# Autodesk Inventor assembly: Conjunto
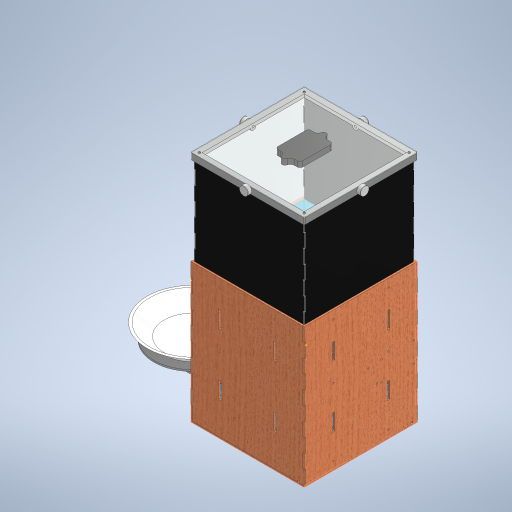
[picture p0: Inventor's stored thumbnail of the model, 512x512]
Saved by Autodesk Inventor 2024.2 (Build 282272000, 272)
## iProperties
Created: 2024-07-16
Part Number: Conjunto
Document SubType Name: Assembly
Designer: sergi
Author: sergi
## Documents named in this file (35)
- C:\Users\sergi\OneDrive\Escritorio\Projects\Automatic Feeder\ComederoV6\Inventor\Conjunto.iam
- C:\Users\sergi\OneDrive\Escritorio\Projects\Automatic Feeder\ComederoV6\Inventor\Contenedor.ipt
- C:\Users\sergi\OneDrive\Escritorio\Projects\Automatic Feeder\ComederoV6\Inventor\Contenedor_Pared_1.ipt
- C:\Users\sergi\OneDrive\Escritorio\Projects\Automatic Feeder\ComederoV6\Inventor\Tolva.ipt
- C:\Users\sergi\OneDrive\Escritorio\Projects\Automatic Feeder\ComederoV6\Inventor\Rodamiento.ipt
- C:\Users\sergi\OneDrive\Escritorio\Projects\Automatic Feeder\ComederoV6\Inventor\Brida_Rodamiento.ipt
- C:\Users\sergi\OneDrive\Escritorio\Projects\Automatic Feeder\ComederoV6\Inventor\Celda_Carga.ipt
- C:\Users\sergi\OneDrive\Escritorio\Projects\Automatic Feeder\ComederoV6\Inventor\Envolvente.ipt
- C:\Users\sergi\OneDrive\Escritorio\Projects\Automatic Feeder\ComederoV6\Inventor\Envolvente_Pared_1.ipt
- C:\Users\sergi\OneDrive\Escritorio\Projects\Automatic Feeder\ComederoV6\Inventor\Soporte_Dosificador.ipt
- C:\Users\sergi\OneDrive\Escritorio\Projects\Automatic Feeder\ComederoV6\Inventor\Brida_Rodamiento_Inferior.ipt
- C:\Users\sergi\OneDrive\Escritorio\Projects\Automatic Feeder\ComederoV6\Inventor\Tope_Dosificador.ipt
- C:\Users\sergi\OneDrive\Escritorio\Projects\Automatic Feeder\ComederoV6\Inventor\Contrapeso.ipt
- C:\Users\sergi\OneDrive\Escritorio\Projects\Automatic Feeder\ComederoV6\Inventor\Cemento.ipt
- C:\Users\sergi\OneDrive\Escritorio\Projects\Automatic Feeder\ComederoV6\Inventor\Tapa_Inferior.ipt
- C:\Users\sergi\OneDrive\Escritorio\Projects\Automatic Feeder\ComederoV6\Inventor\Union_Inferior.ipt
- C:\Users\sergi\OneDrive\Escritorio\Projects\Automatic Feeder\ComederoV6\Inventor\Envolvente_Pared_2.ipt
- C:\Users\sergi\OneDrive\Escritorio\Projects\Automatic Feeder\ComederoV6\Inventor\Rampa_Salida.ipt
- C:\Users\sergi\OneDrive\Escritorio\Projects\Automatic Feeder\ComederoV6\Inventor\Soporte_Cuenco.ipt
- C:\Users\sergi\OneDrive\Escritorio\Projects\Automatic Feeder\ComederoV6\Inventor\Cuenco.ipt
- C:\Users\sergi\OneDrive\Escritorio\Projects\Automatic Feeder\ComederoV6\Inventor\Base_Plato.ipt
- C:\Users\sergi\OneDrive\Escritorio\Projects\Automatic Feeder\ComederoV6\Inventor\Aspas.ipt
- C:\Users\sergi\OneDrive\Escritorio\Projects\Automatic Feeder\ComederoV6\Inventor\Tapadera.ipt
- C:\Users\sergi\OneDrive\Escritorio\Projects\Automatic Feeder\ComederoV6\Inventor\Marco_Tapa.ipt
- C:\Users\sergi\OneDrive\Escritorio\Projects\Automatic Feeder\ComederoV6\Inventor\Deshumidicador.ipt
- C:\Users\sergi\OneDrive\Escritorio\Projects\Automatic Feeder\ComederoV6\Inventor\Servomotor.ipt
- C:\Users\sergi\OneDrive\Escritorio\Projects\Automatic Feeder\ComederoV6\Inventor\Engranajes.iam
- C:\Users\sergi\OneDrive\Escritorio\Projects\Automatic Feeder\ComederoV6\Inventor\Gears\Design Accelerator\Soporte_Servo.ipt
- C:\Users\sergi\OneDrive\Escritorio\Projects\Automatic Feeder\ComederoV6\Inventor\Cabeza_Tornillos.ipt
- C:\Users\sergi\OneDrive\Escritorio\Projects\Automatic Feeder\ComederoV6\Inventor\Tapa_Cabeza_Tornillo.ipt
- C:\Users\sergi\OneDrive\Escritorio\Projects\Automatic Feeder\ComederoV6\Inventor\ESP32S3.ipt
- C:\Users\sergi\OneDrive\Escritorio\Projects\Automatic Feeder\ComederoV6\Inventor\Soporte_ESP32S3.ipt
- C:\Users\sergi\OneDrive\Escritorio\Projects\Automatic Feeder\ComederoV6\Inventor\Buck.ipt
- C:\Users\sergi\OneDrive\Escritorio\Projects\Automatic Feeder\ComederoV6\Inventor\Envolvente_Pared_Trasera.ipt
- C:\Users\sergi\OneDrive\Escritorio\Projects\Automatic Feeder\ComederoV6\Inventor\Envolvente_Pared_Derecha.ipt
## Components (59 placed, 34 different names)
1. Contenedor:1 — Nivelación:1
2. Contenedor_Pared_1:1 — Nivelación:1, Coincidencia:1, Nivelación:2, Nivelación:3, Nivelación:43
3. Contenedor_Pared_1:2 — Coincidencia:1, Nivelación:2, Nivelación:3, Nivelación:6, Coincidencia:3, Nivelación:7, Nivelación:8, Nivelación:13
4. Contenedor_Pared_1:3 — Nivelación:4, Nivelación:6, Coincidencia:3, Nivelación:7
5. Contenedor_Pared_1:4 — Nivelación:4
6. Tolva:1 — Nivelación:8, Coincidencia:4, Coincidencia:5, Nivelación:9, Coincidencia:78
7. Rodamiento:1 — Coincidencia:4, Coincidencia:5
8. Brida_Rodamiento:1 — Nivelación:9, Coincidencia:77
9. Celda_Carga:1 — Coincidencia:67, Coincidencia:70, Coincidencia:72, Coincidencia:74
10. Rodamiento:2 — Coincidencia:37
11. Envolvente:1 — Nivelación:13
12. Envolvente_Pared_1:2 — Coincidencia:13
13. Soporte_Dosificador:1 — Coincidencia:30, Coincidencia:35, Coincidencia:38, Coincidencia:39, Coincidencia:42, Coincidencia:43, Coincidencia:44, Coincidencia:45, Coincidencia:50, Coincidencia:51, Nivelación:30, Nivelación:31, Ángulo:1, Coincidencia:80, Coincidencia:81, Coincidencia:82, Coincidencia:83
14. Tope_Dosificador:1
15. Contrapeso:1 — Coincidencia:27, Coincidencia:28, Coincidencia:29, Coincidencia:33
16. Cemento:1 — Coincidencia:27, Coincidencia:28, Coincidencia:29
17. Tapa_Inferior:1 — Nivelación:27, Coincidencia:12, Coincidencia:14, Coincidencia:17, Coincidencia:18, Coincidencia:21, Coincidencia:22, Coincidencia:23, Coincidencia:24, Coincidencia:25, Coincidencia:26, Nivelación:28, Nivelación:29, Coincidencia:32, Coincidencia:33, Coincidencia:52, Coincidencia:53, Coincidencia:54, Coincidencia:55, Coincidencia:56, Coincidencia:57, Coincidencia:58, Coincidencia:59, Coincidencia:73, Ángulo:2, Coincidencia:100, Nivelación:100, Nivelación:101, Nivelación:102, Nivelación:103
18. Union_Inferior:1 — Nivelación:27
19. Union_Inferior:2 — Coincidencia:12, Coincidencia:13, Coincidencia:14
20. Union_Inferior:3 — Coincidencia:17, Coincidencia:32
21. Union_Inferior:4 — Coincidencia:18
22. Union_Inferior:5 — Coincidencia:22, Coincidencia:103
23. Union_Inferior:6 — Coincidencia:23, Coincidencia:26, Nivelación:28
24. Union_Inferior:7 — Coincidencia:21
25. Union_Inferior:8 — Coincidencia:24, Coincidencia:25, Nivelación:29
26. Brida_Rodamiento_Inferior:1 — Coincidencia:30, Coincidencia:35, Coincidencia:37
27. Union_Inferior:9 — Coincidencia:45, Coincidencia:55
28. Union_Inferior:10 — Coincidencia:51, Coincidencia:56
29. Union_Inferior:11 — Coincidencia:39, Coincidencia:53
30. Union_Inferior:12 — Coincidencia:38, Coincidencia:52, Coincidencia:97
31. Union_Inferior:13 — Coincidencia:44, Coincidencia:54
32. Union_Inferior:14 — Coincidencia:50, Coincidencia:57
33. Union_Inferior:15 — Coincidencia:42, Nivelación:31, Coincidencia:59
34. Union_Inferior:16 — Coincidencia:43, Nivelación:30, Coincidencia:58
35. Envolvente_Pared_2:1 — Nivelación:38, Nivelación:39, Nivelación:40, Coincidencia:65, Coincidencia:66, Coincidencia:73
36. Rampa_Salida:1 — Nivelación:38, Nivelación:39
37. Soporte_Cuenco:1 — Nivelación:40, Coincidencia:61, Coincidencia:72, Coincidencia:74
38. Cuenco:1 — Coincidencia:61, Coincidencia:65, Coincidencia:66, Coincidencia:67, Coincidencia:68, Coincidencia:69
39. Base_Plato:1 — Coincidencia:68, Coincidencia:69, Coincidencia:70
40. Aspas:1
41. Tapadera:1 — Coincidencia:75, Nivelación:44
42. Marco_Tapa:1 — Nivelación:43, Coincidencia:75, Coincidencia:84, Coincidencia:85, Coincidencia:86, Coincidencia:87, Coincidencia:89, Coincidencia:90, Coincidencia:91, Coincidencia:92
43. Deshumidicador:1 — Nivelación:44
44. Servomotor:1 — Coincidencia:79, Ángulo:1
45. Engranajes:1 [sub-assembly] — Coincidencia:77, Coincidencia:78, Coincidencia:79, Coincidencia:80
46. Soporte_Servo:1 — Coincidencia:81, Coincidencia:82, Coincidencia:83
47. Cabeza_Tornillos:1 — Nivelación:45, Coincidencia:84, Coincidencia:85
48. Tapa_Cabeza_Tornillo:1 — Nivelación:45
49. Cabeza_Tornillos:2 — Coincidencia:86, Coincidencia:87, Coincidencia:88
50. Tapa_Cabeza_Tornillo:2 — Coincidencia:88
51. Cabeza_Tornillos:3 — Coincidencia:91, Coincidencia:92, Coincidencia:93
52. Tapa_Cabeza_Tornillo:3 — Coincidencia:93
53. Cabeza_Tornillos:4 — Coincidencia:89, Coincidencia:90, Coincidencia:94, Coincidencia:95
54. Tapa_Cabeza_Tornillo:4 — Coincidencia:94, Coincidencia:95
55. ESP32S3:1 — Nivelación:49
56. Soporte_ESP32S3:1 — Nivelación:49, Coincidencia:97, Coincidencia:99, Nivelación:99, Coincidencia:101
57. Buck:1 — Ángulo:2, Coincidencia:99, Nivelación:99, Coincidencia:102
58. Envolvente_Pared_Trasera:1 — Coincidencia:100, Nivelación:100, Nivelación:101, Coincidencia:101, Coincidencia:102
59. Envolvente_Pared_Derecha:1 — Coincidencia:103, Nivelación:102, Nivelación:103
## Relationships (108: Mate 76, Flush 30, Angle 2)
- Nivelación:1 [Flush]: Contenedor:1 ↔ Contenedor_Pared_1:1
- Coincidencia:1 [Mate]: Contenedor_Pared_1:1 ↔ Contenedor_Pared_1:2
- Nivelación:2 [Flush]: Contenedor_Pared_1:1 ↔ Contenedor_Pared_1:2
- Nivelación:3 [Flush]: Contenedor_Pared_1:1 ↔ Contenedor_Pared_1:2
- [Mate]: Contenedor_Pared_1:3 ↔ Contenedor_Pared_1:4
- Nivelación:4 [Flush]: Contenedor_Pared_1:3 ↔ Contenedor_Pared_1:4
- [Flush]: Contenedor_Pared_1:3 ↔ Contenedor_Pared_1:4
- Nivelación:6 [Flush]: Contenedor_Pared_1:2 ↔ Contenedor_Pared_1:3
- Coincidencia:3 [Mate]: Contenedor_Pared_1:2 ↔ Contenedor_Pared_1:3
- Nivelación:7 [Flush]: Contenedor_Pared_1:2 ↔ Contenedor_Pared_1:3
- Nivelación:8 [Flush]: Contenedor_Pared_1:2 ↔ Tolva:1
- Coincidencia:4 [Mate]: Tolva:1 ↔ Rodamiento:1
- Coincidencia:5 [Mate]: Tolva:1 ↔ Rodamiento:1
- Nivelación:9 [Flush]: Tolva:1 ↔ Brida_Rodamiento:1
- Nivelación:13 [Flush]: Contenedor_Pared_1:2 ↔ Envolvente:1
- Nivelación:27 [Flush]: Tapa_Inferior:1 ↔ Union_Inferior:1
- Coincidencia:12 [Mate]: Tapa_Inferior:1 ↔ Union_Inferior:2
- Coincidencia:13 [Mate]: Envolvente_Pared_1:2 ↔ Union_Inferior:2
- Coincidencia:14 [Mate]: Tapa_Inferior:1 ↔ Union_Inferior:2
- Coincidencia:17 [Mate]: Tapa_Inferior:1 ↔ Union_Inferior:3
- Coincidencia:18 [Mate]: Tapa_Inferior:1 ↔ Union_Inferior:4
- Coincidencia:21 [Mate]: Tapa_Inferior:1 ↔ Union_Inferior:7
- Coincidencia:22 [Mate]: Tapa_Inferior:1 ↔ Union_Inferior:5
- Coincidencia:23 [Mate]: Tapa_Inferior:1 ↔ Union_Inferior:6
- Coincidencia:24 [Mate]: Tapa_Inferior:1 ↔ Union_Inferior:8
- Coincidencia:25 [Mate]: Tapa_Inferior:1 ↔ Union_Inferior:8
- Coincidencia:26 [Mate]: Tapa_Inferior:1 ↔ Union_Inferior:6
- Nivelación:28 [Flush] (3 mm): Tapa_Inferior:1 ↔ Union_Inferior:6
- Nivelación:29 [Flush] (3 mm): Tapa_Inferior:1 ↔ Union_Inferior:8
- Coincidencia:27 [Mate]: Contrapeso:1 ↔ Cemento:1
- Coincidencia:28 [Mate]: Contrapeso:1 ↔ Cemento:1
- Coincidencia:29 [Mate]: Contrapeso:1 ↔ Cemento:1
- Coincidencia:30 [Mate]: Soporte_Dosificador:1 ↔ Brida_Rodamiento_Inferior:1
- Coincidencia:32 [Mate]: Tapa_Inferior:1 ↔ Union_Inferior:3
- Coincidencia:33 [Mate]: Contrapeso:1 ↔ Tapa_Inferior:1
- Coincidencia:35 [Mate]: Soporte_Dosificador:1 ↔ Brida_Rodamiento_Inferior:1
- Coincidencia:37 [Mate]: Rodamiento:2 ↔ Brida_Rodamiento_Inferior:1
- Coincidencia:38 [Mate]: Soporte_Dosificador:1 ↔ Union_Inferior:12
- Coincidencia:39 [Mate]: Soporte_Dosificador:1 ↔ Union_Inferior:11
- Coincidencia:42 [Mate]: Soporte_Dosificador:1 ↔ Union_Inferior:15
- Coincidencia:43 [Mate]: Soporte_Dosificador:1 ↔ Union_Inferior:16
- Coincidencia:44 [Mate]: Soporte_Dosificador:1 ↔ Union_Inferior:13
- Coincidencia:45 [Mate]: Soporte_Dosificador:1 ↔ Union_Inferior:9
- Coincidencia:50 [Mate]: Soporte_Dosificador:1 ↔ Union_Inferior:14
- Coincidencia:51 [Mate]: Soporte_Dosificador:1 ↔ Union_Inferior:10
- Coincidencia:52 [Mate]: Tapa_Inferior:1 ↔ Union_Inferior:12
- Coincidencia:53 [Mate]: Tapa_Inferior:1 ↔ Union_Inferior:11
- Coincidencia:54 [Mate]: Tapa_Inferior:1 ↔ Union_Inferior:13
- Coincidencia:55 [Mate]: Tapa_Inferior:1 ↔ Union_Inferior:9
- Coincidencia:56 [Mate]: Tapa_Inferior:1 ↔ Union_Inferior:10
- Coincidencia:57 [Mate]: Tapa_Inferior:1 ↔ Union_Inferior:14
- Nivelación:30 [Flush]: Soporte_Dosificador:1 ↔ Union_Inferior:16
- Nivelación:31 [Flush]: Soporte_Dosificador:1 ↔ Union_Inferior:15
- Coincidencia:58 [Mate]: Tapa_Inferior:1 ↔ Union_Inferior:16
- Coincidencia:59 [Mate]: Tapa_Inferior:1 ↔ Union_Inferior:15
- Nivelación:38 [Flush]: Envolvente_Pared_2:1 ↔ Rampa_Salida:1
- Nivelación:39 [Flush]: Envolvente_Pared_2:1 ↔ Rampa_Salida:1
- Nivelación:40 [Flush]: Envolvente_Pared_2:1 ↔ Soporte_Cuenco:1
- Coincidencia:61 [Mate]: Soporte_Cuenco:1 ↔ Cuenco:1
- Coincidencia:65 [Mate] (100 mm): Envolvente_Pared_2:1 ↔ Cuenco:1
- Coincidencia:66 [Mate] (-103 mm): Envolvente_Pared_2:1 ↔ Cuenco:1
- Coincidencia:67 [Mate]: Celda_Carga:1 ↔ Cuenco:1
- Coincidencia:68 [Mate]: Cuenco:1 ↔ Base_Plato:1
- Coincidencia:69 [Mate]: Cuenco:1 ↔ Base_Plato:1
- Coincidencia:70 [Mate]: Celda_Carga:1 ↔ Base_Plato:1
- Coincidencia:72 [Mate] (20.05 mm): Celda_Carga:1 ↔ Soporte_Cuenco:1
- Coincidencia:73 [Mate]: Tapa_Inferior:1 ↔ Envolvente_Pared_2:1
- Coincidencia:74 [Mate]: Celda_Carga:1 ↔ Soporte_Cuenco:1
- Nivelación:43 [Flush]: Contenedor_Pared_1:1 ↔ Marco_Tapa:1
- Coincidencia:75 [Mate]: Tapadera:1 ↔ Marco_Tapa:1
- Nivelación:44 [Flush]: Tapadera:1 ↔ Deshumidicador:1
- Coincidencia:77 [Mate]: Brida_Rodamiento:1 ↔ Engranajes:1
- Coincidencia:78 [Mate] (2 mm): Tolva:1 ↔ Engranajes:1
- Coincidencia:79 [Mate]: Servomotor:1 ↔ Engranajes:1
- Ángulo:1 [Angle] (0 deg): Soporte_Dosificador:1 ↔ Servomotor:1
- Coincidencia:80 [Mate]: Soporte_Dosificador:1 ↔ Engranajes:1
- Coincidencia:81 [Mate]: Soporte_Dosificador:1 ↔ Soporte_Servo:1
- Coincidencia:82 [Mate]: Soporte_Dosificador:1 ↔ Soporte_Servo:1
- Coincidencia:83 [Mate]: Soporte_Dosificador:1 ↔ Soporte_Servo:1
- Nivelación:45 [Flush]: Cabeza_Tornillos:1 ↔ Tapa_Cabeza_Tornillo:1
- [Flush]: Cabeza_Tornillos:2 ↔ Tapa_Cabeza_Tornillo:2
- [Flush]: Cabeza_Tornillos:3 ↔ Tapa_Cabeza_Tornillo:3
- [Flush]: Cabeza_Tornillos:4 ↔ Tapa_Cabeza_Tornillo:4
- Coincidencia:84 [Mate]: Marco_Tapa:1 ↔ Cabeza_Tornillos:1
- Coincidencia:85 [Mate]: Marco_Tapa:1 ↔ Cabeza_Tornillos:1
- Coincidencia:86 [Mate]: Marco_Tapa:1 ↔ Cabeza_Tornillos:2
- Coincidencia:87 [Mate]: Marco_Tapa:1 ↔ Cabeza_Tornillos:2
- Coincidencia:88 [Mate]: Cabeza_Tornillos:2 ↔ Tapa_Cabeza_Tornillo:2
- Coincidencia:89 [Mate]: Marco_Tapa:1 ↔ Cabeza_Tornillos:4
- Coincidencia:90 [Mate]: Marco_Tapa:1 ↔ Cabeza_Tornillos:4
- Coincidencia:91 [Mate]: Marco_Tapa:1 ↔ Cabeza_Tornillos:3
- Coincidencia:92 [Mate]: Marco_Tapa:1 ↔ Cabeza_Tornillos:3
- Coincidencia:93 [Mate]: Cabeza_Tornillos:3 ↔ Tapa_Cabeza_Tornillo:3
- Coincidencia:94 [Mate]: Cabeza_Tornillos:4 ↔ Tapa_Cabeza_Tornillo:4
- Coincidencia:95 [Mate]: Cabeza_Tornillos:4 ↔ Tapa_Cabeza_Tornillo:4
- Nivelación:49 [Flush]: ESP32S3:1 ↔ Soporte_ESP32S3:1
- Coincidencia:97 [Mate] (3 mm): Union_Inferior:12 ↔ Soporte_ESP32S3:1
- Ángulo:2 [Angle] (0 deg): Tapa_Inferior:1 ↔ Buck:1
- Coincidencia:99 [Mate] (2 mm): Soporte_ESP32S3:1 ↔ Buck:1
- Nivelación:99 [Flush] (-5 mm): Soporte_ESP32S3:1 ↔ Buck:1
- Coincidencia:100 [Mate]: Tapa_Inferior:1 ↔ Envolvente_Pared_Trasera:1
- Nivelación:100 [Flush]: Tapa_Inferior:1 ↔ Envolvente_Pared_Trasera:1
- Nivelación:101 [Flush]: Tapa_Inferior:1 ↔ Envolvente_Pared_Trasera:1
- Coincidencia:101 [Mate]: Soporte_ESP32S3:1 ↔ Envolvente_Pared_Trasera:1
- Coincidencia:102 [Mate]: Buck:1 ↔ Envolvente_Pared_Trasera:1
- Coincidencia:103 [Mate]: Union_Inferior:5 ↔ Envolvente_Pared_Derecha:1
- Nivelación:102 [Flush]: Tapa_Inferior:1 ↔ Envolvente_Pared_Derecha:1
- Nivelación:103 [Flush]: Tapa_Inferior:1 ↔ Envolvente_Pared_Derecha:1
## Named parameters: d4_d1 = 0 mm, d5_d2 = 0 mm, d6_d3 = 0 mm, d171_d170 = 0 mm, d172_d170 = 0 mm, d173_d170 = 0 mm
